# Autodesk Inventor assembly: 1073 rller
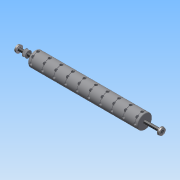
[picture p0: Inventor's stored thumbnail of the model, 180x180]
Saved by Autodesk Inventor 2015 (Build 190159000, 159)
## iProperties
Created: 2017-01-20
Part Number: 1073 rller
Document SubType Name: Assembly
Designer: nick pc
Author: nick pc
## Documents named in this file (5)
- D:\robotics\1073 rller.iam
- D:\robotics\Imported Components\thunder hex\thunder hex.ipt
- D:\robotics\BRUCES ROLLER.ipt
- D:\robotics\Imported Components\.5 HEX BEARING\.5 HEX BEARING.ipt
- D:\robotics\test belt sprocket.ipt
## Components (5 placed, 4 different names)
1. thunder hex:1 — Rigid:1, Rotational:1, Rotational:2
2. BRUCES ROLLER:1 — Rigid:1
3. .5 HEX BEARING:1 — Rotational:1
4. .5 HEX BEARING:2 — Rotational:2, Rotational:3
5. test belt sprocket:1 — Rotational:3
## Relationships (4: RevoluteJoint 3, WeldJoint 1)
- Rigid:1 [WeldJoint] (-76.2 mm): thunder hex:1 ↔ BRUCES ROLLER:1
- Rotational:1 [RevoluteJoint]: thunder hex:1 ↔ .5 HEX BEARING:1
- Rotational:2 [RevoluteJoint] (7.62 mm): thunder hex:1 ↔ .5 HEX BEARING:2
- Rotational:3 [RevoluteJoint] (25.4 mm): .5 HEX BEARING:2 ↔ test belt sprocket:1
